# Autodesk Inventor assembly: Monitor_Blanking_V3
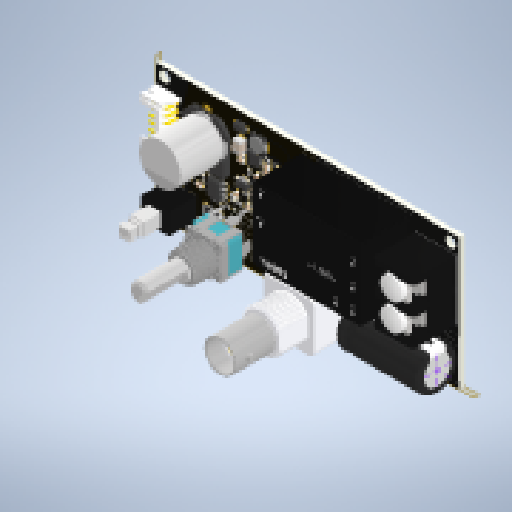
[picture p0: Inventor's stored thumbnail of the model, 512x512]
Saved by Autodesk Inventor 2025.3 (Build 293356000, 356)
## iProperties
Created: 2025-06-10
Part Number: Monitor_Blanking_V3
Document SubType Name: Assembly
Designer: Yuhsuan Chen
Author: Yuhsuan Chen
## Documents named in this file (44)
- C:\Users\Yuhsuan Chen\Desktop\ME\Monitor blanking\Source\PCBA\Monitor_Blanking_V3.iam
- C:\Users\Yuhsuan Chen\Desktop\ME\Monitor blanking\Source\PCBA\Monitor_Blanking_V3_BOARD.ipt
- C:\Users\Yuhsuan Chen\Desktop\ME\Monitor blanking\Source\PCBA\ConvertedComponents\CAP_CHIP_0603_CMP-611-0050-6.ipt
- C:\Users\Yuhsuan Chen\Desktop\ME\Monitor blanking\Source\PCBA\ConvertedComponents\WSON6_CMP-970-0077-1.ipt
- C:\Users\Yuhsuan Chen\Desktop\ME\Monitor blanking\Source\PCBA\ConvertedComponents\RES_CHIP_0603_CMP-633-0052-25.ipt
- C:\Users\Yuhsuan Chen\Desktop\ME\Monitor blanking\Source\PCBA\ConvertedComponents\RES_CHIP_0603_CMP-633-0070-21.ipt
- C:\Users\Yuhsuan Chen\Desktop\ME\Monitor blanking\Source\PCBA\ConvertedComponents\RES_CHIP_0603_CMP-633-0002-26.ipt
- C:\Users\Yuhsuan Chen\Desktop\ME\Monitor blanking\Source\PCBA\ConvertedComponents\RES_CHIP_0603_CMP-633-0119-5.ipt
- C:\Users\Yuhsuan Chen\Desktop\ME\Monitor blanking\Source\PCBA\ConvertedComponents\RES_CHIP_0603_CMP-633-0169-1.ipt
- C:\Users\Yuhsuan Chen\Desktop\ME\Monitor blanking\Source\PCBA\ConvertedComponents\QFN16_3X3_0.5E_EP_CMP-970-0074-1.ipt
- C:\Users\Yuhsuan Chen\Desktop\ME\Monitor blanking\Source\PCBA\ConvertedComponents\CAP_CHIP_1210_CMP-611-0087-1.ipt
- C:\Users\Yuhsuan Chen\Desktop\ME\Monitor blanking\Source\PCBA\ConvertedComponents\CAP_CHIP_0603_CMP-611-0088-1.ipt
- C:\Users\Yuhsuan Chen\Desktop\ME\Monitor blanking\Source\PCBA\ConvertedComponents\ECAP_SMD_D12.5_13.5L_CMP-612-0011-1.ipt
- C:\Users\Yuhsuan Chen\Desktop\ME\Monitor blanking\Source\PCBA\ConvertedComponents\TUHS15F12_CMP-A10-0017-1.ipt
- C:\Users\Yuhsuan Chen\Desktop\ME\Monitor blanking\Source\PCBA\ConvertedComponents\RES_CHIP_0603_CMP-633-0073-25.ipt
- C:\Users\Yuhsuan Chen\Desktop\ME\Monitor blanking\Source\PCBA\ConvertedComponents\RES_CHIP_2010_CMP-633-0165-2.ipt
- C:\Users\Yuhsuan Chen\Desktop\ME\Monitor blanking\Source\PCBA\ConvertedComponents\CAP_CHIP_0603_CMP-611-0027-24.ipt
- C:\Users\Yuhsuan Chen\Desktop\ME\Monitor blanking\Source\PCBA\ConvertedComponents\SOIC8_CMP-941-0015-1.ipt
- C:\Users\Yuhsuan Chen\Desktop\ME\Monitor blanking\Source\PCBA\ConvertedComponents\SOT23-5_CMP-970-0038-1.ipt
- C:\Users\Yuhsuan Chen\Desktop\ME\Monitor blanking\Source\PCBA\ConvertedComponents\SOT23-5_CMP-970-0067-1.ipt
- C:\Users\Yuhsuan Chen\Desktop\ME\Monitor blanking\Source\PCBA\ConvertedComponents\RES_CHIP_0603_CMP-633-0013-26.ipt
- C:\Users\Yuhsuan Chen\Desktop\ME\Monitor blanking\Source\PCBA\ConvertedComponents\RES_CHIP_0603_CMP-633-0143-1.ipt
- C:\Users\Yuhsuan Chen\Desktop\ME\Monitor blanking\Source\PCBA\ConvertedComponents\CAP_CHIP_0603_CMP-611-0033-11.ipt
- C:\Users\Yuhsuan Chen\Desktop\ME\Monitor blanking\Source\PCBA\ConvertedComponents\SW_LOCK_SPPH410100_CMP-B00-0031-1.ipt
- C:\Users\Yuhsuan Chen\Desktop\ME\Monitor blanking\Source\PCBA\ConvertedComponents\SOT23-5_CMP-970-0051-1.ipt
- C:\Users\Yuhsuan Chen\Desktop\ME\Monitor blanking\Source\PCBA\ConvertedComponents\RES_CHIP_2010_CMP-633-0149-2.ipt
- C:\Users\Yuhsuan Chen\Desktop\ME\Monitor blanking\Source\PCBA\ConvertedComponents\RES_CHIP_0603_CMP-633-0167-1.ipt
- C:\Users\Yuhsuan Chen\Desktop\ME\Monitor blanking\Source\PCBA\ConvertedComponents\RES_CHIP_0603_CMP-633-0000-28.ipt
- C:\Users\Yuhsuan Chen\Desktop\ME\Monitor blanking\Source\PCBA\ConvertedComponents\RES_CHIP_0603_CMP-633-0118-5.ipt
- C:\Users\Yuhsuan Chen\Desktop\ME\Monitor blanking\Source\PCBA\ConvertedComponents\RK09L1140_CMP-632-0008-2.ipt
- C:\Users\Yuhsuan Chen\Desktop\ME\Monitor blanking\Source\PCBA\ConvertedComponents\SOT23_CMP-810-0002-2.ipt
- C:\Users\Yuhsuan Chen\Desktop\ME\Monitor blanking\Source\PCBA\ConvertedComponents\TDSON-8_CMP-830-0011-2.ipt
- C:\Users\Yuhsuan Chen\Desktop\ME\Monitor blanking\Source\PCBA\ConvertedComponents\IND_PWR_0404_CMP-620-0021-1.ipt
- C:\Users\Yuhsuan Chen\Desktop\ME\Monitor blanking\Source\PCBA\ConvertedComponents\SOD123_CMP-821-0014-1.ipt
- C:\Users\Yuhsuan Chen\Desktop\ME\Monitor blanking\Source\PCBA\ConvertedComponents\PH_DIP_90_1X6P_CMP-370-0048-1.ipt
- C:\Users\Yuhsuan Chen\Desktop\ME\Monitor blanking\Source\PCBA\ConvertedComponents\BT-8.26-1X2P_CMP-330-0001-1.ipt
- C:\Users\Yuhsuan Chen\Desktop\ME\Monitor blanking\Source\PCBA\ConvertedComponents\CAP_CHIP_0603_CMP-611-0022-7.ipt
- C:\Users\Yuhsuan Chen\Desktop\ME\Monitor blanking\Source\PCBA\ConvertedComponents\CAP_CHIP_0603_CMP-611-0085-1.ipt
- C:\Users\Yuhsuan Chen\Desktop\ME\Monitor blanking\Source\PCBA\ConvertedComponents\CAP_CHIP_0603_CMP-611-0076-2.ipt
- C:\Users\Yuhsuan Chen\Desktop\ME\Monitor blanking\Source\PCBA\ConvertedComponents\ECAP_DIP_12.5_90_CMP-612-0013-1.ipt
- C:\Users\Yuhsuan Chen\Desktop\ME\Monitor blanking\Source\PCBA\ConvertedComponents\SO5_CMP-530-0005-1.ipt
- C:\Users\Yuhsuan Chen\Desktop\ME\Monitor blanking\Source\PCBA\ConvertedComponents\RES_CHIP_0603_CMP-633-0020-24.ipt
- C:\Users\Yuhsuan Chen\Desktop\ME\Monitor blanking\Source\PCBA\ConvertedComponents\BNC-TE-5227222_CMP-730-0010-3.ipt
- C:\Users\Yuhsuan Chen\Desktop\ME\Monitor blanking\Source\RING.ipt
## Components (63 placed, 63 different names)
1. Monitor_Blanking_V3_BOARD:1 — Mate:2
2. CAP_CHIP_0603_CMP-611-0050-6:1{C11}
3. CAP_CHIP_0603_CMP-611-0050-6:2{C13}
4. CAP_CHIP_0603_CMP-611-0050-6:3{C14}
5. WSON6_CMP-970-0077-1:1{U4}
6. RES_CHIP_0603_CMP-633-0052-25:1{R15}
7. RES_CHIP_0603_CMP-633-0052-25:2{R17}
8. RES_CHIP_0603_CMP-633-0070-21:1{R14}
9. RES_CHIP_0603_CMP-633-0002-26:1{R13}
10. RES_CHIP_0603_CMP-633-0002-26:2{R23}
11. RES_CHIP_0603_CMP-633-0002-26:3{R2}
12. RES_CHIP_0603_CMP-633-0002-26:4{R9}
13. RES_CHIP_0603_CMP-633-0119-5:1{R12}
14. RES_CHIP_0603_CMP-633-0169-1:1{R11}
15. QFN16_3X3_0.5E_EP_CMP-970-0074-1:1{U3}
16. CAP_CHIP_1210_CMP-611-0087-1:1{C7}
17. CAP_CHIP_0603_CMP-611-0088-1:1{C6}
18. ECAP_SMD_D12.5_13.5L_CMP-612-0011-1:1{C3}
19. TUHS15F12_CMP-A10-0017-1:1{U1}
20. RES_CHIP_0603_CMP-633-0073-25:1{R22}
21. RES_CHIP_2010_CMP-633-0165-2:1{R1}
22. CAP_CHIP_0603_CMP-611-0027-24:1{C22}
23. CAP_CHIP_0603_CMP-611-0027-24:2{C21}
24. CAP_CHIP_0603_CMP-611-0027-24:3{C19}
25. CAP_CHIP_0603_CMP-611-0027-24:4{C8}
26. CAP_CHIP_0603_CMP-611-0027-24:5{C1}
27. SOIC8_CMP-941-0015-1:1{U8}
28. SOT23-5_CMP-970-0038-1:1{U5}
29. SOT23-5_CMP-970-0067-1:1{U6}
30. RES_CHIP_0603_CMP-633-0013-26:1{R18}
31. RES_CHIP_0603_CMP-633-0013-26:2{R10}
32. RES_CHIP_0603_CMP-633-0013-26:3{R20}
33. RES_CHIP_0603_CMP-633-0013-26:4{R19}
34. RES_CHIP_0603_CMP-633-0013-26:5{R6}
35. RES_CHIP_0603_CMP-633-0143-1:1{R16}
36. CAP_CHIP_0603_CMP-611-0033-11:1{C18}
37. CAP_CHIP_0603_CMP-611-0033-11:2{C12}
38. CAP_CHIP_0603_CMP-611-0033-11:3{C17}
39. CAP_CHIP_0603_CMP-611-0033-11:4{C16}
40. CAP_CHIP_0603_CMP-611-0033-11:5{C15}
41. CAP_CHIP_0603_CMP-611-0033-11:6{C5}
42. CAP_CHIP_0603_CMP-611-0033-11:7{C4}
43. SW_LOCK_SPPH410100_CMP-B00-0031-1:1{SW1}
44. SOT23-5_CMP-970-0051-1:1{U7}
45. RES_CHIP_2010_CMP-633-0149-2:1{R21}
46. RES_CHIP_0603_CMP-633-0167-1:1{R8}
47. RES_CHIP_0603_CMP-633-0000-28:1{R7}
48. RES_CHIP_0603_CMP-633-0118-5:1{R5}
49. RK09L1140_CMP-632-0008-2:1{R3} — Mate:3, Mate:4
50. SOT23_CMP-810-0002-2:1{Q2}
51. TDSON-8_CMP-830-0011-2:1{Q1}
52. IND_PWR_0404_CMP-620-0021-1:1{L1}
53. SOD123_CMP-821-0014-1:1{D1}
54. PH_DIP_90_1X6P_CMP-370-0048-1:1{CN2}
55. BT-8.26-1X2P_CMP-330-0001-1:1{CN1}
56. CAP_CHIP_0603_CMP-611-0022-7:1{C20}
57. CAP_CHIP_0603_CMP-611-0085-1:1{C10}
58. CAP_CHIP_0603_CMP-611-0076-2:1{C9}
59. ECAP_DIP_12.5_90_CMP-612-0013-1:1{C2}
60. SO5_CMP-530-0005-1:1{U2}
61. RES_CHIP_0603_CMP-633-0020-24:1{R4}
62. BNC-TE-5227222_CMP-730-0010-3:1{CN3}
63. RING:1 — Mate:2, Mate:3, Mate:4
## Relationships (3: Mate 3)
- Mate:2: Monitor_Blanking_V3_BOARD:1 ↔ RING:1
- Mate:3: RK09L1140_CMP-632-0008-2:1{R3} ↔ RING:1
- Mate:4: RK09L1140_CMP-632-0008-2:1{R3} ↔ RING:1
